# Autodesk Inventor assembly: D5MG
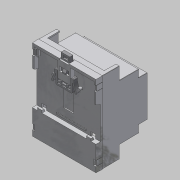
[picture p0: Inventor's stored thumbnail of the model, 180x180]
Saved by Autodesk Inventor 2018 (Build 220112000, 112)
## iProperties
Created: 2017-08-14
Part Number: D5MG
Material: Типовые
Document SubType Name: Assembly
Designer: shawn
Author: shawn
## Documents named in this file (6)
- D:\Abbath\03 RaceIt WorkSpace\Библиотеки\!3D модели\Корпуса приборные\Gainta\D4MG\3D\Inv\D4MG.iam
- D4MG.iam
- D:\Abbath\03 RaceIt WorkSpace\Библиотеки\!3D модели\Корпуса приборные\Gainta\D4MG\3D\Inv\D4MG-BASE.ipt
- D:\Abbath\03 RaceIt WorkSpace\Библиотеки\!3D модели\Корпуса приборные\Gainta\D4MG\3D\Inv\D4MG-BODY.ipt
- D:\Abbath\03 RaceIt WorkSpace\Библиотеки\!3D модели\Корпуса приборные\Gainta\D4MG\3D\Inv\D4MG-COVER.ipt
- D:\Abbath\03 RaceIt WorkSpace\Библиотеки\!3D модели\Корпуса приборные\Gainta\D4MG\3D\Inv\D4MG-WALL CLIP.ipt
## Components (4 placed, 4 different names)
1. D4MG-BASE:1 — Совмещение:1, Совмещение:2, Совмещение:3, Совмещение:5
2. D4MG-BODY:1 — Совмещение:1, Совмещение:2, Совмещение:3, Совмещение:4
3. D4MG-COVER:1 — Совмещение:4
4. D4MG-WALL CLIP:1 — Совмещение:5
## Relationships (5: Mate 5)
- Совмещение:1 [Mate]: D4MG-BASE:1 ↔ D4MG-BODY:1
- Совмещение:2 [Mate]: D4MG-BASE:1 ↔ D4MG-BODY:1
- Совмещение:3 [Mate]: D4MG-BASE:1 ↔ D4MG-BODY:1
- Совмещение:4 [Mate]: D4MG-BODY:1 ↔ D4MG-COVER:1
- Совмещение:5 [Mate]: D4MG-BASE:1 ↔ D4MG-WALL CLIP:1
